# Autodesk Inventor assembly: anglechangefinal
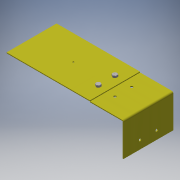
[picture p0: Inventor's stored thumbnail of the model, 180x180]
Saved by Autodesk Inventor 2019 (Build 230136000, 136)
## iProperties
Created: 2020-02-15
Part Number: anglechangefinal
Document SubType Name: Assembly
Designer: Dell
Author: Dell
## Documents named in this file (5)
- C:\Users\Dell\Documents\anglechangefinal.iam
- C:\Users\Dell\Documents\anglechange.ipt
- C:\Users\Dell\Documents\clamp.ipt
- C:\Users\Dell\Documents\nut2.ipt
- C:\Users\Dell\Documents\bolt.ipt
## Components (6 placed, 4 different names)
1. anglechange:1 — Rotational:1, Rotational:2, Rotational:3
2. clamp:1 — Rotational:1, Rotational:4, Rotational:5
3. nut2:1 — Rotational:5
4. nut2:2 — Rotational:4
5. bolt:1 — Rotational:2
6. bolt:2 — Rotational:3
## Relationships (5: RevoluteJoint 5)
- Rotational:1 [RevoluteJoint]: anglechange:1 ↔ clamp:1
- Rotational:2 [RevoluteJoint]: anglechange:1 ↔ bolt:1
- Rotational:3 [RevoluteJoint]: anglechange:1 ↔ bolt:2
- Rotational:4 [RevoluteJoint]: clamp:1 ↔ nut2:2
- Rotational:5 [RevoluteJoint]: clamp:1 ↔ nut2:1
